# Autodesk Inventor assembly: Idler Stack
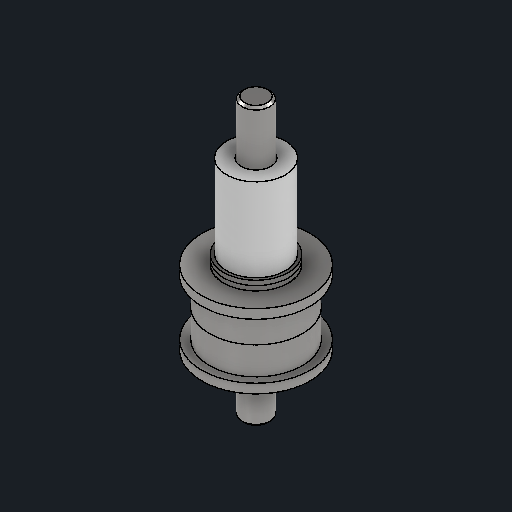
[picture p0: Inventor's stored thumbnail of the model, 512x512]
Saved by Autodesk Inventor 2026.1 (Build 301233020, 233B)
## iProperties
Created: 2025-08-01
Part Number: Idler Stack
Document SubType Name: Assembly
Designer: Joshua Eah
Author: Joshua Eah
## Documents named in this file (5)
- C:\Users\JoshuaEah\Documents\GitHub\Voron-0\CAD\X Axis\XY Joints\XY Joint Left\Left Idler Stack.iam
- C:\Users\JoshuaEah\Documents\GitHub\Voron-0\CAD\Hardware\3x30 Pin.ipt
- C:\Users\JoshuaEah\Documents\GitHub\Voron-0\CAD\Hardware\Bearings\F623 Stack.iam
- C:\Users\JoshuaEah\Documents\GitHub\Voron-0\CAD\X Axis\XY Joints\Spacer\Spacer.ipt
- C:\Users\JoshuaEah\Documents\GitHub\Voron-0\CAD\Hardware\Fasteners\M3_Washer.ipt
## Components (5 placed, 4 different names)
1. 3x30 Pin:1
2. F623 Stack:1 [sub-assembly]
3. Spacer:1
4. M3_Washer:1
5. M3_Washer:2
## Relationships (4: Insert 3, Mate 1)
- [Insert]: F623 Stack:1 ↔ M3_Washer:1
- [Insert]: F623 Stack:1 ↔ M3_Washer:2
- [Mate]: 3x30 Pin:1 ↔ F623 Stack:1
- [Insert]: Spacer:1 ↔ M3_Washer:2
